# Autodesk Inventor assembly: Ensamblaje2
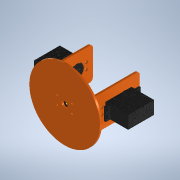
[picture p0: Inventor's stored thumbnail of the model, 180x180]
Saved by Autodesk Inventor 2021 (Build 250183000, 183)
## iProperties
Created: 2021-04-02
Part Number: Ensamblaje2
Document SubType Name: Assembly
Designer: diego
Author: diego
## Documents named in this file (5)
- C:\Users\diego\Desktop\Diego\Utadeo 2021-1\Robotica Industrial\Corte 2\Solido planos\Ensamblaje2.iam
- C:\Users\diego\Desktop\Diego\Utadeo 2021-1\Robotica Industrial\Corte 2\Solido planos\Base2.ipt
- C:\Users\diego\Desktop\Diego\Utadeo 2021-1\Robotica Industrial\Corte 2\Solido planos\7.ipt
- C:\Users\diego\Desktop\Diego\Utadeo 2021-1\Robotica Industrial\Corte 2\Solido planos\Extension2.ipt
- C:\Users\diego\Desktop\Diego\Utadeo 2021-1\Robotica Industrial\Corte 2\Solido planos\Servo.ipt
## Components (5 placed, 4 different names)
1. Base2:1 — Coincidencia:1, Coincidencia:2
2. Extension2:1 — Coincidencia:1, Coincidencia:2, Coincidencia:3
3. 7:1 — Coincidencia:3, De rotación:1, De rotación:2
4. Servo:1 — De rotación:1
5. Servo:2 — De rotación:2
## Relationships (5: Mate 3, RevoluteJoint 2)
- Coincidencia:1 [Mate]: Base2:1 ↔ Extension2:1
- Coincidencia:2 [Mate]: Base2:1 ↔ Extension2:1
- Coincidencia:3 [Mate]: Extension2:1 ↔ 7:1
- De rotación:1 [RevoluteJoint] (3 mm): 7:1 ↔ Servo:1
- De rotación:2 [RevoluteJoint] (-3 mm): 7:1 ↔ Servo:2
